# Autodesk Inventor assembly: AMR
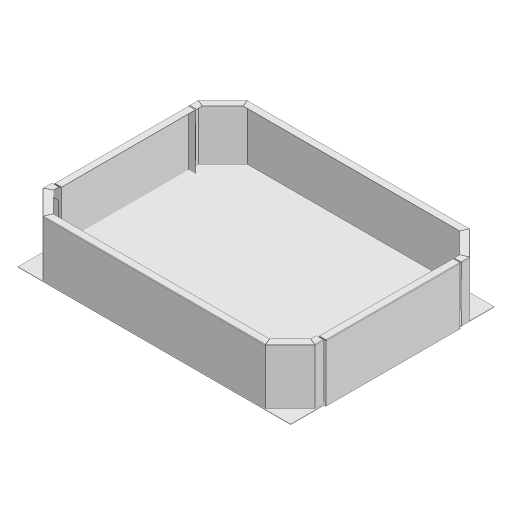
[picture p0: Inventor's stored thumbnail of the model, 512x512]
Saved by Autodesk Inventor 2024.2 (Build 282272000, 272)
## iProperties
Created: 2025-01-06
Part Number: AMR
Document SubType Name: Assembly
Designer: Kartik
Mass: 961.963 g
Surface Area: 19601.7 cm^2
Volume: 961.963 cm^3
Density: 1 g/cm^3
Author: Kartik
## Documents named in this file (6)
- D:\Kartik\AMR\Custom_Design\Assembly\AMR.iam
- D:\Kartik\AMR\Custom_Design\Parts\Back_plate.ipt
- D:\Kartik\AMR\Custom_Design\Parts\Base_Plate.ipt
- D:\Kartik\AMR\Custom_Design\Parts\Front_plate.ipt
- D:\Kartik\AMR\Custom_Design\Parts\Side_plate_1.ipt
- D:\Kartik\AMR\Custom_Design\Parts\Side_plate_2.ipt
## Components (5 placed, 5 different names)
1. Back_plate:1 — Flush:3, Flush:4, Flush:5, Mate:2, Flush:6
2. Base_Plate:1 — Mate:3, Mate:4, Mate:5
3. Front_plate:1 — Flush:1, Flush:2, Mate:1, Flush:5, Mate:5
4. Side_plate_1:1 — Flush:1, Flush:2, Mate:1, Flush:3, Flush:4, Mate:3, Mate:4
5. Side_plate_2:1 — Mate:2, Flush:6
## Relationships (11: Flush 6, Mate 5)
- Flush:1: Front_plate:1 ↔ Side_plate_1:1
- Flush:2: Front_plate:1 ↔ Side_plate_1:1
- Mate:1 (1 mm): Front_plate:1 ↔ Side_plate_1:1
- Flush:3: Back_plate:1 ↔ Side_plate_1:1
- Flush:4: Back_plate:1 ↔ Side_plate_1:1
- Flush:5: Back_plate:1 ↔ Front_plate:1
- Mate:2 (1 mm): Back_plate:1 ↔ Side_plate_2:1
- Flush:6: Back_plate:1 ↔ Side_plate_2:1
- Mate:3: Base_Plate:1 ↔ Side_plate_1:1
- Mate:4: Base_Plate:1 ↔ Side_plate_1:1
- Mate:5: Base_Plate:1 ↔ Front_plate:1
